# Autodesk Inventor assembly: LeftUpperArm
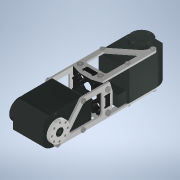
[picture p0: Inventor's stored thumbnail of the model, 180x180]
Saved by Autodesk Inventor 2020.4 (Build 244396000, 396)
## iProperties
Created: 2021-09-11
Part Number: LeftUpperArm
Document SubType Name: Assembly
Designer: Masato
Author: Masato
## Documents named in this file (8)
- C:\Users\Masato\Documents\Inventor\CIT Brains_Inventor\OpenPlatform_ver3_0（ワッシャ変更）\UpperBody\Arm\LeftUpperArm.iam
- C:\Users\Masato\Documents\Inventor\CIT Brains_Inventor\OpenPlatform_ver3_0（ワッシャ変更）\UpperBody\Arm\UpperArm_side_frame.ipt
- C:\Users\Masato\Documents\Inventor\CIT Brains_Inventor\OpenPlatform_ver3_0（ワッシャ変更）\UpperBody\Arm\UpperArm_diagonal.ipt
- C:\Users\Masato\Documents\Inventor\CIT Brains_Inventor\OpenPlatform_ver3_0（ワッシャ変更）\Ready_Made\B3M10xx.ipt
- C:\Users\Masato\Documents\Inventor\CIT Brains_Inventor\OpenPlatform_ver3_0（ワッシャ変更）\Ready_Made\FreeHorn.ipt
- C:\Users\Masato\Documents\Inventor\CIT Brains_Inventor\OpenPlatform_ver3_0（ワッシャ変更）\Ready_Made\Screw\M2_6-15.ipt
- C:\Users\Masato\Documents\Inventor\CIT Brains_Inventor\OpenPlatform_ver3_0（ワッシャ変更）\Ready_Made\Screw\M2_6-20.ipt
- C:\Users\Masato\Documents\Inventor\CIT Brains_Inventor\OpenPlatform_ver3_0（ワッシャ変更）\Ready_Made\Screw\M3-6.ipt
## Components (29 placed, 7 different names)
1. UpperArm_diagonal:1 — 挿入:46, 挿入:47, 挿入:62, 挿入:63
2. B3M10xx:1 — 挿入:22, 挿入:23, 挿入:24, 挿入:25, 挿入:26, 挿入:30, 挿入:31, 挿入:32
3. B3M10xx:2 — 挿入:21, 挿入:36, 挿入:37, 挿入:38, 挿入:56, 挿入:57, 挿入:58
4. FreeHorn:1 — 挿入:22
5. FreeHorn:2 — 挿入:21
6. M2_6-15:1 — 挿入:29
7. M2_6-15:2 — 挿入:27
8. M2_6-15:3 — 挿入:28
9. M2_6-15:4 — 挿入:43
10. M2_6-15:5 — 挿入:44
11. M2_6-15:6 — 挿入:45
12. M2_6-20:1 — 挿入:33
13. M2_6-20:2 — 挿入:35
14. M2_6-20:3 — 挿入:34
15. M2_6-20:4 — 挿入:59
16. M2_6-20:5 — 挿入:60
17. M2_6-20:6 — 挿入:61
18. M3-6:1 — 挿入:55
19. M3-6:2 — 挿入:54
20. M3-6:3 — 挿入:51
21. M3-6:4 — 挿入:50
22. M3-6:5 — 挿入:41
23. M3-6:6 — 挿入:42
24. M3-6:7 — 挿入:49
25. M3-6:8 — 挿入:48
26. UpperArm_side_frame:1 — 挿入:54, 挿入:55, 挿入:56, 挿入:57, 挿入:58, 挿入:59, 挿入:60, 挿入:61, 挿入:63
27. UpperArm_side_frame:2 — 挿入:36, 挿入:37, 挿入:38, 挿入:41, 挿入:42, 挿入:43, 挿入:44, 挿入:45, 挿入:62
28. UpperArm_side_frame:3 — 挿入:30, 挿入:31, 挿入:32, 挿入:33, 挿入:34, 挿入:35, 挿入:50, 挿入:51
29. UpperArm_side_frame:4 — 挿入:23, 挿入:24, 挿入:25, 挿入:26, 挿入:27, 挿入:28, 挿入:29, 挿入:46, 挿入:47, 挿入:48, 挿入:49
## Relationships (39: Insert 39)
- 挿入:21 [Insert]: B3M10xx:2 ↔ FreeHorn:2
- 挿入:22 [Insert]: B3M10xx:1 ↔ FreeHorn:1
- 挿入:23 [Insert]: B3M10xx:1 ↔ UpperArm_side_frame:4
- 挿入:24 [Insert]: B3M10xx:1 ↔ UpperArm_side_frame:4
- 挿入:25 [Insert]: B3M10xx:1 ↔ UpperArm_side_frame:4
- 挿入:26 [Insert]: B3M10xx:1 ↔ UpperArm_side_frame:4
- 挿入:27 [Insert]: M2_6-15:2 ↔ UpperArm_side_frame:4
- 挿入:28 [Insert]: M2_6-15:3 ↔ UpperArm_side_frame:4
- 挿入:29 [Insert]: M2_6-15:1 ↔ UpperArm_side_frame:4
- 挿入:30 [Insert]: B3M10xx:1 ↔ UpperArm_side_frame:3
- 挿入:31 [Insert]: B3M10xx:1 ↔ UpperArm_side_frame:3
- 挿入:32 [Insert]: B3M10xx:1 ↔ UpperArm_side_frame:3
- 挿入:33 [Insert]: M2_6-20:1 ↔ UpperArm_side_frame:3
- 挿入:34 [Insert]: M2_6-20:3 ↔ UpperArm_side_frame:3
- 挿入:35 [Insert]: M2_6-20:2 ↔ UpperArm_side_frame:3
- 挿入:36 [Insert]: B3M10xx:2 ↔ UpperArm_side_frame:2
- 挿入:37 [Insert]: B3M10xx:2 ↔ UpperArm_side_frame:2
- 挿入:38 [Insert]: B3M10xx:2 ↔ UpperArm_side_frame:2
- 挿入:41 [Insert]: M3-6:5 ↔ UpperArm_side_frame:2
- 挿入:42 [Insert]: M3-6:6 ↔ UpperArm_side_frame:2
- 挿入:43 [Insert]: M2_6-15:4 ↔ UpperArm_side_frame:2
- 挿入:44 [Insert]: M2_6-15:5 ↔ UpperArm_side_frame:2
- 挿入:45 [Insert]: M2_6-15:6 ↔ UpperArm_side_frame:2
- 挿入:46 [Insert]: UpperArm_diagonal:1 ↔ UpperArm_side_frame:4
- 挿入:47 [Insert]: UpperArm_diagonal:1 ↔ UpperArm_side_frame:4
- 挿入:48 [Insert]: M3-6:8 ↔ UpperArm_side_frame:4
- 挿入:49 [Insert]: M3-6:7 ↔ UpperArm_side_frame:4
- 挿入:50 [Insert]: M3-6:4 ↔ UpperArm_side_frame:3
- 挿入:51 [Insert]: M3-6:3 ↔ UpperArm_side_frame:3
- 挿入:54 [Insert]: M3-6:2 ↔ UpperArm_side_frame:1
- 挿入:55 [Insert]: M3-6:1 ↔ UpperArm_side_frame:1
- 挿入:56 [Insert]: B3M10xx:2 ↔ UpperArm_side_frame:1
- 挿入:57 [Insert]: B3M10xx:2 ↔ UpperArm_side_frame:1
- 挿入:58 [Insert]: B3M10xx:2 ↔ UpperArm_side_frame:1
- 挿入:59 [Insert]: M2_6-20:4 ↔ UpperArm_side_frame:1
- 挿入:60 [Insert]: M2_6-20:5 ↔ UpperArm_side_frame:1
- 挿入:61 [Insert]: M2_6-20:6 ↔ UpperArm_side_frame:1
- 挿入:62 [Insert]: UpperArm_diagonal:1 ↔ UpperArm_side_frame:2
- 挿入:63 [Insert]: UpperArm_diagonal:1 ↔ UpperArm_side_frame:1
